# Autodesk Inventor assembly: СОВЕРШЕНСТВО без говна_MIR
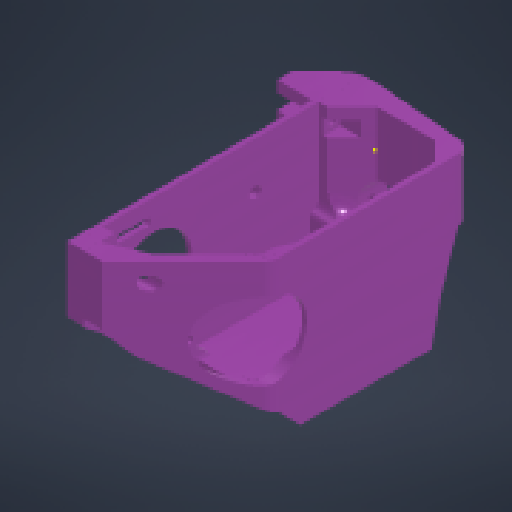
[picture p0: Inventor's stored thumbnail of the model, 512x512]
Saved by Autodesk Inventor 2025 (Build 290162000, 162)
## iProperties
Created: 2024-10-08
Part Number: СОВЕРШЕНСТВО без говна_MIR
Document SubType Name: Assembly
Designer: Phantom
Mass: 291.072 g
Surface Area: 978.884 cm^2
Volume: 188.885 cm^3
Density: 1.541 g/cm^3
Author: Phantom
## Documents named in this file (3)
- C:\Users\Phantom\Desktop\Phantom16950\СОВЕРШЕНСТВО без говна_MIR.iam
- C:\Users\Phantom\Desktop\Phantom16950\репление колёс СОВЕРШЕННОЕ ТОЛСТАЯ_MIR.ipt
- C:\Users\Phantom\Desktop\Phantom16950\репление колёс СОВЕРШЕННОЕ ТОНКАЯ_MIR.ipt
## Components (2 placed, 2 different names)
1. репление колёс СОВЕРШЕННОЕ ТОЛСТАЯ_MIR:1 — Совмещение:2, Заподлицо:1, Совмещение:1
2. репление колёс СОВЕРШЕННОЕ ТОНКАЯ_MIR:1 — Совмещение:2, Заподлицо:1, Совмещение:1
## Relationships (3: Mate 2, Flush 1)
- Совмещение:2 [Mate]: репление колёс СОВЕРШЕННОЕ ТОЛСТАЯ_MIR:1 ↔ репление колёс СОВЕРШЕННОЕ ТОНКАЯ_MIR:1
- Заподлицо:1 [Flush]: репление колёс СОВЕРШЕННОЕ ТОЛСТАЯ_MIR:1 ↔ репление колёс СОВЕРШЕННОЕ ТОНКАЯ_MIR:1
- Совмещение:1 [Mate]: репление колёс СОВЕРШЕННОЕ ТОЛСТАЯ_MIR:1 ↔ репление колёс СОВЕРШЕННОЕ ТОНКАЯ_MIR:1
